# Autodesk Inventor assembly: maszt final final
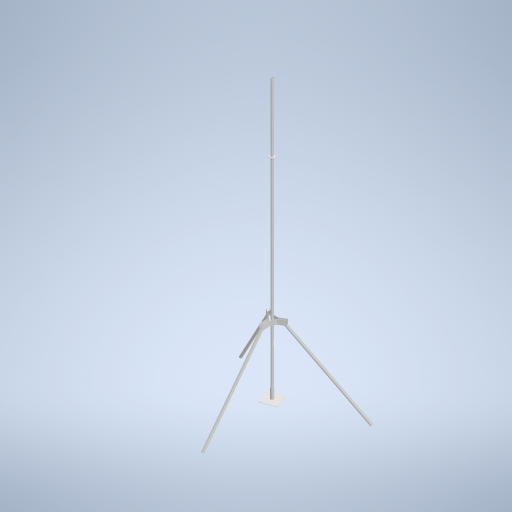
[picture p0: Inventor's stored thumbnail of the model, 512x512]
Saved by Autodesk Inventor 2024 (Build 280153000, 153)
## iProperties
Created: 2024-11-18
Part Number: maszt final final
Document SubType Name: Assembly
Designer: Admin
Author: Admin
## Documents named in this file (10)
- C:\Users\Karolina\OneDrive\Pulpit\R7_STR_9000_MastGS\R7_STR_9000_MastGS.iam
- C:\Users\Karolina\OneDrive\Pulpit\R7_STR_9000_MastGS\R7_STR_9001_mast.ipt
- C:\Users\Karolina\OneDrive\Pulpit\R7_STR_9000_MastGS\R7_STR_9005_clamp.ipt
- C:\Users\x\Desktop\Nowy folder\tuleja dystansowa.ipt
- C:\Users\Karolina\OneDrive\Pulpit\R7_STR_9000_MastGS\R7_STR_9004_branches.ipt
- C:\Users\Karolina\OneDrive\Pulpit\R7_STR_9000_MastGS\R7_STR_9003_tube_stand.ipt
- C:\Users\Karolina\OneDrive\Pulpit\R7_STR_9000_MastGS\R7_STR_9002_sheet_Al.ipt
- C:\Users\Karolina\OneDrive\Pulpit\R7_STR_9000_MastGS\R7_STR_9006_mast2_wires.ipt
- C:\Users\Karolina\OneDrive\Pulpit\R7_STR_9000_MastGS\R7_STR_9010_plyta2.ipt
- C:\Users\Karolina\OneDrive\Pulpit\R7_STR_9000_MastGS\R7_STR_9007_sheet_wires.ipt
## Components (22 placed, 9 different names)
1. R7_STR_9005_clamp:1 — Rotational:5
2. R7_STR_9005_clamp:2 — Rigid:5, Rigid:6, Rotational:2, Rigid:7
3. R7_STR_9005_clamp:3 — Rigid:8, Rotational:3, Rotational:4
4. tuleja dystansowa:1 — Rotational:2, Rigid:8
5. tuleja dystansowa:2 — Rigid:6
6. tuleja dystansowa:3 — Rotational:4
7. tuleja dystansowa:4 — Rigid:7
8. tuleja dystansowa:5 — Rotational:3, Rotational:5
9. tuleja dystansowa:6 — Rigid:5
10. R7_STR_9001_mast:1 — Rotational:9, Insert:2
11. R7_STR_9001_mast:3
12. R7_STR_9001_mast:4 — Rotational:8, Rotational:9
13. R7_STR_9001_mast:5 — Rotational:7, Rotational:8
14. R7_STR_9001_mast:6 — Rotational:7, Insert:1
15. R7_STR_9004_branches:2
16. R7_STR_9004_branches:4
17. R7_STR_9004_branches:5
18. R7_STR_9003_tube_stand:1 — Insert:1, Rigid:9
19. R7_STR_9002_sheet_Al:1 — Rigid:9
20. R7_STR_9006_mast2_wires:1 — Insert:2, Rigid:10
21. R7_STR_9010_plyta2:1 — Rigid:10, Rotational:10
22. R7_STR_9007_sheet_wires:1 — Rotational:10
## Relationships (16: RevoluteJoint 8, WeldJoint 6, Insert 2)
- Rigid:5 [WeldJoint]: R7_STR_9005_clamp:2 ↔ tuleja dystansowa:6
- Rigid:6 [WeldJoint]: R7_STR_9005_clamp:2 ↔ tuleja dystansowa:2
- Rotational:2 [RevoluteJoint]: R7_STR_9005_clamp:2 ↔ tuleja dystansowa:1
- Rigid:7 [WeldJoint]: R7_STR_9005_clamp:2 ↔ tuleja dystansowa:4
- Rigid:8 [WeldJoint]: R7_STR_9005_clamp:3 ↔ tuleja dystansowa:1
- Rotational:3 [RevoluteJoint]: R7_STR_9005_clamp:3 ↔ tuleja dystansowa:5
- Rotational:4 [RevoluteJoint]: R7_STR_9005_clamp:3 ↔ tuleja dystansowa:3
- Rotational:5 [RevoluteJoint]: R7_STR_9005_clamp:1 ↔ tuleja dystansowa:5
- Rotational:7 [RevoluteJoint]: R7_STR_9001_mast:5 ↔ R7_STR_9001_mast:6
- Rotational:8 [RevoluteJoint]: R7_STR_9001_mast:4 ↔ R7_STR_9001_mast:5
- Rotational:9 [RevoluteJoint]: R7_STR_9001_mast:1 ↔ R7_STR_9001_mast:4
- Insert:1: R7_STR_9001_mast:6 ↔ R7_STR_9003_tube_stand:1
- Rigid:9 [WeldJoint]: R7_STR_9003_tube_stand:1 ↔ R7_STR_9002_sheet_Al:1
- Insert:2: R7_STR_9001_mast:1 ↔ R7_STR_9006_mast2_wires:1
- Rigid:10 [WeldJoint]: R7_STR_9006_mast2_wires:1 ↔ R7_STR_9010_plyta2:1
- Rotational:10 [RevoluteJoint]: R7_STR_9010_plyta2:1 ↔ R7_STR_9007_sheet_wires:1
